# Autodesk Inventor assembly: Assembly
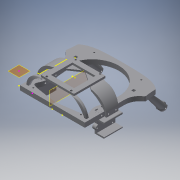
[picture p0: Inventor's stored thumbnail of the model, 180x180]
Saved by Autodesk Inventor 2019 (Build 230136000, 136)
## iProperties
Created: 2019-04-08
Part Number: Assembly
Material: Ogólny
Document SubType Name: Assembly
Designer: terg
Author: terg
## Documents named in this file (7)
- D:\Projekt\Projekt---platforma-mobilna\Chassis\Assembly.iam
- D:\Projekt\Projekt---platforma-mobilna\Chassis\base.ipt
- D:\Projekt\Projekt---platforma-mobilna\Chassis\motor_grip_L.ipt
- D:\Projekt\Projekt---platforma-mobilna\Chassis\motor_grip_R.ipt
- D:\Projekt\Projekt---platforma-mobilna\Chassis\wheel.ipt
- D:\Projekt\Projekt---platforma-mobilna\Chassis\cpu_grip.ipt
- D:\Projekt\Projekt---platforma-mobilna\Chassis\cpu_grip_2.ipt
## Components (7 placed, 6 different names)
1. base:1 — Płaskie:1, Płaskie:2, Obrotowe:1, Obrotowe:2, Zestawiający:1, Zestawiający:2, Sztywne:1, Obrotowe:3
2. motor_grip_L:1 — Płaskie:1
3. motor_grip_R:1 — Płaskie:2
4. wheel:1 — Obrotowe:2, Zestawiający:1
5. wheel:2 — Obrotowe:1, Zestawiający:2
6. cpu_grip:1 — Sztywne:1
7. cpu_grip_2:1 — Obrotowe:3
## Relationships (8: RevoluteJoint 3, PlanarJoint 2, Mate 2, WeldJoint 1)
- Płaskie:1 [PlanarJoint]: base:1 ↔ motor_grip_L:1
- Płaskie:2 [PlanarJoint]: base:1 ↔ motor_grip_R:1
- Obrotowe:1 [RevoluteJoint] (1 mm): base:1 ↔ wheel:2
- Obrotowe:2 [RevoluteJoint] (-1 mm): base:1 ↔ wheel:1
- Zestawiający:1 [Mate]: base:1 ↔ wheel:1
- Zestawiający:2 [Mate]: base:1 ↔ wheel:2
- Sztywne:1 [WeldJoint]: base:1 ↔ cpu_grip:1
- Obrotowe:3 [RevoluteJoint] (-1.3 mm): base:1 ↔ cpu_grip_2:1
